# Autodesk Inventor assembly: flipper_tank_assembly
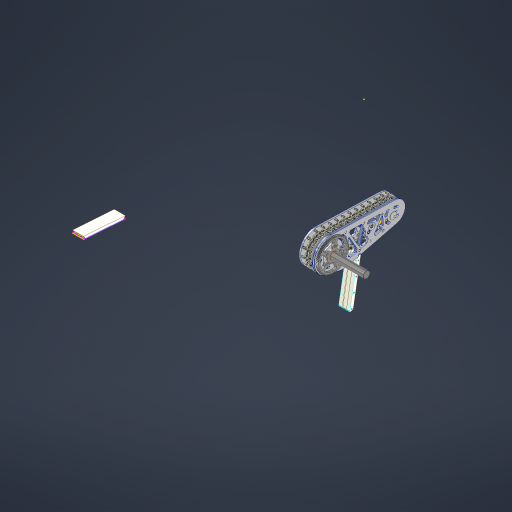
[picture p0: Inventor's stored thumbnail of the model, 512x512]
Saved by Autodesk Inventor 2023.2 (Build 272271030, 271C)
## iProperties
Created: 2023-02-28
Part Number: flipper_tank_assembly
Document SubType Name: Assembly
Designer: ralph
Author: ralph
## Documents named in this file (20)
- C:\Users\ralph\OneDrive\Documents\GrabCAD\Robocup Rescue\Drive\v1\TANK flipper\flipper_tank_assembly.iam
- C:\Users\ralph\OneDrive\Documents\GrabCAD\Robocup Rescue\Drive\v1\TANK flipper\single tank.ipt
- C:\Users\ralph\OneDrive\Documents\GrabCAD\Robocup Rescue\Drive\v1\TANK flipper\Drive Shaft.ipt
- C:\Users\ralph\OneDrive\Documents\GrabCAD\Robocup Rescue\Drive\v1\TANK flipper\98585A121_Heavy Duty External Retaining Ring v2(Mirror).ipt
- C:\Users\ralph\OneDrive\Documents\GrabCAD\Robocup Rescue\Drive\v1\TANK flipper\27t track drive sprocket v25.iam
- C:\Users\ralph\OneDrive\Documents\GrabCAD\Robocup Rescue\Drive\v1\TANK flipper\flipper_tensioner.iam
- C:\Users\ralph\OneDrive\Documents\GrabCAD\Robocup Rescue\Drive\v1\TANK flipper\tank_inside_panel.ipt
- C:\Users\ralph\OneDrive\Documents\GrabCAD\Robocup Rescue\Drive\v1\TANK flipper\91263A553_Zinc-Plated Alloy Steel Hex Drive Flat Head Screw v1.ipt
- C:\Users\ralph\OneDrive\Documents\GrabCAD\Robocup Rescue\Drive\v1\TANK flipper\94328A911_Black Oxide Alloy Steel Low-Profile Shoulder Screw v2.ipt
- C:\Users\ralph\OneDrive\Documents\GrabCAD\Robocup Rescue\Drive\v1\TANK flipper\tensioner washer.ipt
- C:\Users\ralph\OneDrive\Documents\GrabCAD\Robocup Rescue\Drive\v1\TANK flipper\chain_female v7.ipt
- C:\Users\ralph\OneDrive\Documents\GrabCAD\Robocup Rescue\Drive\v1\TANK flipper\chain_male v7.ipt
- C:\Users\ralph\OneDrive\Documents\GrabCAD\Robocup Rescue\Drive\v1\TANK flipper\gearSpacer.ipt
- C:\Users\ralph\OneDrive\Documents\GrabCAD\Robocup Rescue\Drive\v1\TANK flipper\Spur Gear (74 teeth).ipt
- C:\Users\ralph\OneDrive\Documents\GrabCAD\Robocup Rescue\Drive\v1\TANK flipper\chain guide.ipt
- C:\Users\ralph\OneDrive\Documents\GrabCAD\Robocup Rescue\Drive\v1\TANK flipper\91253A245_Black-Oxide Alloy Steel Hex Drive Flat Head Screw v1.ipt
- C:\Users\ralph\OneDrive\Documents\GrabCAD\Robocup Rescue\Drive\v1\TANK flipper\flat chain guide.ipt
- C:\Users\ralph\OneDrive\Documents\GrabCAD\Robocup Rescue\Drive\v1\TANK flipper\panel bushing support.ipt
- C:\Users\ralph\OneDrive\Documents\GrabCAD\Robocup Rescue\Drive\v1\TANK flipper\91259A167_Alloy Steel Shoulder Screw\91259A167_Alloy Steel Shoulder Screw.ipt
- C:\Users\ralph\OneDrive\Documents\GrabCAD\Robocup Rescue\Drive\v1\TANK flipper\2868T199_High-Load Oil-Embedded 863 Sleeve Bearing (1) v2(Mirror).ipt
## Components (109 placed, 19 different names)
1. single tank:1 — Rotational:2, Rigid:5, Rigid:8, Rotational:4, Rotational:5, Rotational:6, Rotational:7, Rotational:8, Rotational:9, Rotational:16, Flush:4, Flush:5, Rotational:34, Rotational:35, Rotational:36, Rotational:37, Rotational:45, Rotational:46, Rotational:47, Rotational:51
2. tank_inside_panel:1 — Rotational:10, Rotational:11, Rotational:17, Tangent:1, Tangent:2, Tangent:3, Rigid:12, Flush:6, Flush:7, Flush:8, Flush:9, Rotational:38, Rotational:39, Rotational:40, Rotational:41, Flush:10, Flush:11, Rotational:48, Rotational:49, Rotational:50, Rotational:52
3. Drive Shaft:1 — Rotational:2, Rigid:2, Rigid:3, Rigid:4, Flush:3, Rigid:6
4. 27t track drive sprocket v25:1 [sub-assembly] — Rigid:4, Cylindrical:1, Cylindrical:2, Cylindrical:3, Mate:1
5. gearSpacer:1 — Rigid:12, Rigid:13, Rotational:56, Rotational:58
6. Spur Gear (74 teeth):1 — Rigid:13, Rotational:54, Rotational:55, Rotational:59
7. panel bushing support:1 — Rotational:52, Rotational:57
8. panel bushing support:2 — Rotational:51, Rigid:14
9. 91259A167_Alloy Steel Shoulder Screw:1 — Rotational:54, Rotational:55
10. single tank:2 — Rotational:56
11. 2868T199_High-Load Oil-Embedded 863 Sleeve Bearing (1) v2(Mirror):1 — Rigid:14
12. 2868T199_High-Load Oil-Embedded 863 Sleeve Bearing (1) v2(Mirror):2 — Rotational:58, Rotational:59
13. 2868T199_High-Load Oil-Embedded 863 Sleeve Bearing (1) v2(Mirror):3 — Rotational:57
14. 91263A553_Zinc-Plated Alloy Steel Hex Drive Flat Head Screw v1:3 — Rotational:4
15. 91263A553_Zinc-Plated Alloy Steel Hex Drive Flat Head Screw v1:4 — Rigid:8
16. 91263A553_Zinc-Plated Alloy Steel Hex Drive Flat Head Screw v1:5 — Rotational:5
17. 91263A553_Zinc-Plated Alloy Steel Hex Drive Flat Head Screw v1:9 — Rotational:7
18. 91263A553_Zinc-Plated Alloy Steel Hex Drive Flat Head Screw v1:10 — Rotational:6
19. 94328A911_Black Oxide Alloy Steel Low-Profile Shoulder Screw v2:1 — Rigid:10
20. tensioner washer:1 — Rotational:16, Rigid:10
21. 94328A911_Black Oxide Alloy Steel Low-Profile Shoulder Screw v2:2 — Rigid:11
22. tensioner washer:2 — Rotational:17, Rigid:11
23. flipper_tensioner:1 [sub-assembly] — Rigid:5, Cylindrical:8, Cylindrical:10, Cylindrical:11, Cylindrical:13, Cylindrical:14, Cylindrical:15, Cylindrical:16, Cylindrical:18
24. 91263A553_Zinc-Plated Alloy Steel Hex Drive Flat Head Screw v1:1 — Rotational:9
25. 91263A553_Zinc-Plated Alloy Steel Hex Drive Flat Head Screw v1:12 — Rotational:11
26. 91263A553_Zinc-Plated Alloy Steel Hex Drive Flat Head Screw v1:13 — Rotational:10
27. 91263A553_Zinc-Plated Alloy Steel Hex Drive Flat Head Screw v1:14 — Rotational:8
28. 98585A121_Heavy Duty External Retaining Ring v2(Mirror):1 — Rigid:3
29. 98585A121_Heavy Duty External Retaining Ring v2(Mirror):2 — Rigid:2, Flush:2
30. 98585A121_Heavy Duty External Retaining Ring v2(Mirror):3 — Rigid:6
31. flat chain guide:1 — Flush:10, Flush:11, Mate:2
32. 91253A245_Black-Oxide Alloy Steel Hex Drive Flat Head Screw v1:9 — Rotational:45
33. 91253A245_Black-Oxide Alloy Steel Hex Drive Flat Head Screw v1:10 — Rotational:46
34. 91253A245_Black-Oxide Alloy Steel Hex Drive Flat Head Screw v1:11 — Rotational:47
35. 91253A245_Black-Oxide Alloy Steel Hex Drive Flat Head Screw v1:12 — Rotational:50
36. 91253A245_Black-Oxide Alloy Steel Hex Drive Flat Head Screw v1:13 — Rotational:48
37. 91253A245_Black-Oxide Alloy Steel Hex Drive Flat Head Screw v1:14 — Rotational:49
38. chain guide:1 — Flush:6, Flush:7, Tangent:7
39. 91253A245_Black-Oxide Alloy Steel Hex Drive Flat Head Screw v1:1 — Rotational:34
40. 91253A245_Black-Oxide Alloy Steel Hex Drive Flat Head Screw v1:2 — Rotational:36
41. 91253A245_Black-Oxide Alloy Steel Hex Drive Flat Head Screw v1:3 — Rotational:35
42. 91253A245_Black-Oxide Alloy Steel Hex Drive Flat Head Screw v1:4 — Rotational:37
43. 91253A245_Black-Oxide Alloy Steel Hex Drive Flat Head Screw v1:5 — Rotational:38
44. 91253A245_Black-Oxide Alloy Steel Hex Drive Flat Head Screw v1:6 — Rotational:39
45. 91253A245_Black-Oxide Alloy Steel Hex Drive Flat Head Screw v1:7 — Rotational:40
46. 91253A245_Black-Oxide Alloy Steel Hex Drive Flat Head Screw v1:8 — Rotational:41
47. chain_male v7:37 — Rotational:44, Cylindrical:21
48. chain_female v7:35 — Cylindrical:21
49. chain_male v7:36 — Cylindrical:20, Rotational:43
50. chain_female v7:34 — Rotational:43
51. chain_male v7:34 — Cylindrical:19, Rotational:42
52. chain_female v7:33 — Rotational:42, Cylindrical:20
53. chain_female v7:8 — Rotational:21, Flush:4, Rotational:22
54. chain_male v7:7 — Rotational:20, Rotational:21
55. chain_female v7:6 — Rotational:19, Tangent:1, Tangent:2, Tangent:3, Mate:1, Rotational:20
56. chain_male v7:6 — Cylindrical:4, Rotational:24
57. chain_male v7:30 — Cylindrical:17, Cylindrical:18
58. chain_female v7:29 — Rotational:33, Cylindrical:16, Cylindrical:17
59. chain_female v7:21 — Rotational:24, Flush:8
60. chain_female v7:20 — Flush:9, Cylindrical:19
61. chain_male v7:20 — Rotational:28
62. chain_male v7:32 — Cylindrical:12, Cylindrical:13, Rotational:31
63. chain_female v7:31 — Rotational:30, Cylindrical:11, Cylindrical:12
64. chain_male v7:31 — Rotational:32, Cylindrical:15, Rotational:33
65. chain_female v7:30 — Rotational:31, Cylindrical:14, Rotational:32
66. chain_female v7:32 — Rotational:29, Cylindrical:8, Cylindrical:9
67. chain_male v7:33 — Cylindrical:9, Cylindrical:10, Rotational:30
68. chain_male v7:1 — Rotational:18, Cylindrical:1, Cylindrical:2, Rotational:19
69. chain_female v7:1 — Rotational:18, Cylindrical:3
70. chain_male v7:2
71. chain_female v7:2
72. chain_male v7:3
73. chain_female v7:3
74. chain_male v7:4
75. chain_female v7:4
76. chain_male v7:5
77. chain_female v7:5 — Cylindrical:4
78. chain_female v7:7 — Rotational:23, Flush:5
79. chain_male v7:8 — Rotational:22, Rotational:23
80. chain_female v7:11
81. chain_male v7:12
82. chain_female v7:12
83. chain_male v7:13
84. chain_female v7:13
85. chain_male v7:14
86. chain_female v7:14
87. chain_male v7:15
88. chain_female v7:15 — Mate:2
89. chain_male v7:16
90. chain_female v7:16
91. chain_male v7:17
92. chain_female v7:17 — Rotational:44
93. chain_male v7:18
94. chain_male v7:19 — Cylindrical:7
95. chain_female v7:18 — Rotational:28, Tangent:7, Cylindrical:7
96. chain_male v7:23
97. chain_female v7:22
98. chain_male v7:24
99. chain_female v7:23
100. chain_male v7:25
101. chain_female v7:24
102. chain_male v7:26
103. chain_female v7:25
104. chain_male v7:27
105. chain_female v7:26
106. chain_male v7:28
107. chain_female v7:27
108. chain_male v7:29 — Rotational:29
109. chain_female v7:28
## Component patterns: (5 elements, first: chain_male v7:1 + chain_female v7:1), (8 elements, first: chain_female v7:7 + chain_male v7:8), (8 elements, first: chain_male v7:19 + chain_female v7:18)
## Relationships (95: RevoluteJoint 49, CylindricalJoint 19, WeldJoint 11, Flush 10, Tangent 4, Mate 2)
- Rotational:2 [RevoluteJoint]: single tank:1 ↔ Drive Shaft:1
- Rigid:2 [WeldJoint]: Drive Shaft:1 ↔ 98585A121_Heavy Duty External Retaining Ring v2(Mirror):2
- Rigid:3 [WeldJoint]: Drive Shaft:1 ↔ 98585A121_Heavy Duty External Retaining Ring v2(Mirror):1
- Rigid:4 [WeldJoint]: Drive Shaft:1 ↔ 27t track drive sprocket v25:1
- Rigid:5 [WeldJoint]: single tank:1 ↔ flipper_tensioner:1
- Flush:2 (26.162 mm): 98585A121_Heavy Duty External Retaining Ring v2(Mirror):2
- Flush:3: Drive Shaft:1
- Rigid:6 [WeldJoint]: Drive Shaft:1 ↔ 98585A121_Heavy Duty External Retaining Ring v2(Mirror):3
- Rigid:8 [WeldJoint]: single tank:1 ↔ 91263A553_Zinc-Plated Alloy Steel Hex Drive Flat Head Screw v1:4
- Rotational:4 [RevoluteJoint]: single tank:1 ↔ 91263A553_Zinc-Plated Alloy Steel Hex Drive Flat Head Screw v1:3
- Rotational:5 [RevoluteJoint]: single tank:1 ↔ 91263A553_Zinc-Plated Alloy Steel Hex Drive Flat Head Screw v1:5
- Rotational:6 [RevoluteJoint]: single tank:1 ↔ 91263A553_Zinc-Plated Alloy Steel Hex Drive Flat Head Screw v1:10
- Rotational:7 [RevoluteJoint]: single tank:1 ↔ 91263A553_Zinc-Plated Alloy Steel Hex Drive Flat Head Screw v1:9
- Rotational:8 [RevoluteJoint]: single tank:1 ↔ 91263A553_Zinc-Plated Alloy Steel Hex Drive Flat Head Screw v1:14
- Rotational:9 [RevoluteJoint]: single tank:1 ↔ 91263A553_Zinc-Plated Alloy Steel Hex Drive Flat Head Screw v1:1
- Rotational:10 [RevoluteJoint]: tank_inside_panel:1 ↔ 91263A553_Zinc-Plated Alloy Steel Hex Drive Flat Head Screw v1:13
- Rotational:11 [RevoluteJoint]: tank_inside_panel:1 ↔ 91263A553_Zinc-Plated Alloy Steel Hex Drive Flat Head Screw v1:12
- Rotational:16 [RevoluteJoint]: single tank:1 ↔ tensioner washer:1
- Rotational:17 [RevoluteJoint]: tank_inside_panel:1 ↔ tensioner washer:2
- Rigid:10 [WeldJoint]: 94328A911_Black Oxide Alloy Steel Low-Profile Shoulder Screw v2:1 ↔ tensioner washer:1
- Rigid:11 [WeldJoint]: 94328A911_Black Oxide Alloy Steel Low-Profile Shoulder Screw v2:2 ↔ tensioner washer:2
- Rotational:18 [RevoluteJoint]: chain_male v7:1 ↔ chain_female v7:1
- Cylindrical:1: 27t track drive sprocket v25:1 ↔ chain_male v7:1
- Cylindrical:2: 27t track drive sprocket v25:1 ↔ chain_male v7:1
- Cylindrical:3: 27t track drive sprocket v25:1 ↔ chain_female v7:1
- Cylindrical:4: chain_male v7:6 ↔ chain_female v7:5
- Rotational:19 [RevoluteJoint]: chain_female v7:6 ↔ chain_male v7:1
- Tangent:1: tank_inside_panel:1 ↔ chain_female v7:6
- Tangent:2: tank_inside_panel:1 ↔ chain_female v7:6
- Tangent:3: tank_inside_panel:1 ↔ chain_female v7:6
- Mate:1: 27t track drive sprocket v25:1 ↔ chain_female v7:6
- Rotational:20 [RevoluteJoint]: chain_male v7:7 ↔ chain_female v7:6
- Rotational:21 [RevoluteJoint]: chain_female v7:8 ↔ chain_male v7:7
- Flush:4: single tank:1 ↔ chain_female v7:8
- Rotational:22 [RevoluteJoint]: chain_female v7:8 ↔ chain_male v7:8
- Rotational:23 [RevoluteJoint]: chain_female v7:7 ↔ chain_male v7:8
- Flush:5: single tank:1 ↔ chain_female v7:7
- Rigid:12 [WeldJoint]: tank_inside_panel:1 ↔ gearSpacer:1
- Rigid:13 [WeldJoint]: gearSpacer:1 ↔ Spur Gear (74 teeth):1
- Flush:6: tank_inside_panel:1 ↔ chain guide:1
- Flush:7: tank_inside_panel:1 ↔ chain guide:1
- Rotational:24 [RevoluteJoint]: chain_male v7:6 ↔ chain_female v7:21
- Flush:8: tank_inside_panel:1 ↔ chain_female v7:21
- Flush:9: tank_inside_panel:1 ↔ chain_female v7:20
- Rotational:28 [RevoluteJoint]: chain_male v7:20 ↔ chain_female v7:18
- Tangent:7: chain guide:1 ↔ chain_female v7:18
- Cylindrical:7: chain_male v7:19 ↔ chain_female v7:18
- Rotational:29 [RevoluteJoint]: chain_female v7:32 ↔ chain_male v7:29
- Cylindrical:8: flipper_tensioner:1 ↔ chain_female v7:32
- Cylindrical:9: chain_female v7:32 ↔ chain_male v7:33
- Cylindrical:10: flipper_tensioner:1 ↔ chain_male v7:33
- Rotational:30 [RevoluteJoint]: chain_female v7:31 ↔ chain_male v7:33
- Cylindrical:11: flipper_tensioner:1 ↔ chain_female v7:31
- Cylindrical:12: chain_male v7:32 ↔ chain_female v7:31
- Cylindrical:13: flipper_tensioner:1 ↔ chain_male v7:32
- Rotational:31 [RevoluteJoint]: chain_male v7:32 ↔ chain_female v7:30
- Cylindrical:14: flipper_tensioner:1 ↔ chain_female v7:30
- Rotational:32 [RevoluteJoint]: chain_male v7:31 ↔ chain_female v7:30
- Cylindrical:15: flipper_tensioner:1 ↔ chain_male v7:31
- Rotational:33 [RevoluteJoint]: chain_female v7:29 ↔ chain_male v7:31
- Cylindrical:16: flipper_tensioner:1 ↔ chain_female v7:29
- Cylindrical:17: chain_male v7:30 ↔ chain_female v7:29
- Cylindrical:18: flipper_tensioner:1 ↔ chain_male v7:30
- Rotational:34 [RevoluteJoint]: single tank:1 ↔ 91253A245_Black-Oxide Alloy Steel Hex Drive Flat Head Screw v1:1
- Rotational:35 [RevoluteJoint]: single tank:1 ↔ 91253A245_Black-Oxide Alloy Steel Hex Drive Flat Head Screw v1:3
- Rotational:36 [RevoluteJoint]: single tank:1 ↔ 91253A245_Black-Oxide Alloy Steel Hex Drive Flat Head Screw v1:2
- Rotational:37 [RevoluteJoint]: single tank:1 ↔ 91253A245_Black-Oxide Alloy Steel Hex Drive Flat Head Screw v1:4
- Rotational:38 [RevoluteJoint]: tank_inside_panel:1 ↔ 91253A245_Black-Oxide Alloy Steel Hex Drive Flat Head Screw v1:5
- Rotational:39 [RevoluteJoint]: tank_inside_panel:1 ↔ 91253A245_Black-Oxide Alloy Steel Hex Drive Flat Head Screw v1:6
- Rotational:40 [RevoluteJoint]: tank_inside_panel:1 ↔ 91253A245_Black-Oxide Alloy Steel Hex Drive Flat Head Screw v1:7
- Rotational:41 [RevoluteJoint]: tank_inside_panel:1 ↔ 91253A245_Black-Oxide Alloy Steel Hex Drive Flat Head Screw v1:8
- Cylindrical:19: chain_male v7:34 ↔ chain_female v7:20
- Rotational:42 [RevoluteJoint]: chain_male v7:34 ↔ chain_female v7:33
- Cylindrical:20: chain_male v7:36 ↔ chain_female v7:33
- Rotational:43 [RevoluteJoint]: chain_male v7:36 ↔ chain_female v7:34
- Rotational:44 [RevoluteJoint]: chain_male v7:37 ↔ chain_female v7:17
- Cylindrical:21: chain_male v7:37 ↔ chain_female v7:35
- Flush:10: tank_inside_panel:1 ↔ flat chain guide:1
- Flush:11: tank_inside_panel:1 ↔ flat chain guide:1
- Rotational:45 [RevoluteJoint]: single tank:1 ↔ 91253A245_Black-Oxide Alloy Steel Hex Drive Flat Head Screw v1:9
- Rotational:46 [RevoluteJoint]: single tank:1 ↔ 91253A245_Black-Oxide Alloy Steel Hex Drive Flat Head Screw v1:10
- Rotational:47 [RevoluteJoint]: single tank:1 ↔ 91253A245_Black-Oxide Alloy Steel Hex Drive Flat Head Screw v1:11
- Rotational:48 [RevoluteJoint]: tank_inside_panel:1 ↔ 91253A245_Black-Oxide Alloy Steel Hex Drive Flat Head Screw v1:13
- Rotational:49 [RevoluteJoint]: tank_inside_panel:1 ↔ 91253A245_Black-Oxide Alloy Steel Hex Drive Flat Head Screw v1:14
- Rotational:50 [RevoluteJoint]: tank_inside_panel:1 ↔ 91253A245_Black-Oxide Alloy Steel Hex Drive Flat Head Screw v1:12
- Mate:2: flat chain guide:1 ↔ chain_female v7:15
- Rotational:51 [RevoluteJoint]: single tank:1 ↔ panel bushing support:2
- Rotational:52 [RevoluteJoint]: tank_inside_panel:1 ↔ panel bushing support:1
- Rotational:54 [RevoluteJoint]: Spur Gear (74 teeth):1 ↔ 91259A167_Alloy Steel Shoulder Screw:1
- Rotational:55 [RevoluteJoint]: Spur Gear (74 teeth):1 ↔ 91259A167_Alloy Steel Shoulder Screw:1
- Rotational:56 [RevoluteJoint]: gearSpacer:1 ↔ single tank:2
- Rigid:14 [WeldJoint]: panel bushing support:2 ↔ 2868T199_High-Load Oil-Embedded 863 Sleeve Bearing (1) v2(Mirror):1
- Rotational:57 [RevoluteJoint]: panel bushing support:1 ↔ 2868T199_High-Load Oil-Embedded 863 Sleeve Bearing (1) v2(Mirror):3
- Rotational:58 [RevoluteJoint]: gearSpacer:1 ↔ 2868T199_High-Load Oil-Embedded 863 Sleeve Bearing (1) v2(Mirror):2
- Rotational:59 [RevoluteJoint]: Spur Gear (74 teeth):1 ↔ 2868T199_High-Load Oil-Embedded 863 Sleeve Bearing (1) v2(Mirror):2
